# Autodesk Inventor assembly: FO-020.75-NT
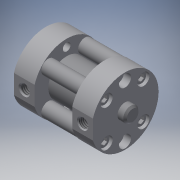
[picture p0: Inventor's stored thumbnail of the model, 180x180]
Saved by Autodesk Inventor 2019.4 (Build 234330000, 330)
## iProperties
Category: PARTsolutions
Company: BIMBA
Created: 2020-02-04
Part Number: FO-020.75-NT
Catalog Web Link: www.cadenas.de
Description: FO, FOD, FOR, FOS-Bimba FLAT-1
Vendor: BIMBA
Document SubType Name: Assembly
Designer: psadmin
Manufacturer: BIMBA
Mass: 12.4329 g
Surface Area: 117.093 cm^2
Volume: 12.4329 cm^3
Density: 1 g/cm^3
PSOL_IDENT_0: {$CADENAS_DATA\23d-libs\bimba\bimba_brand\bimba_imperial\bimba_full_line\flat_cylinders\fo1\bif_asmt
PSOL_IDENT_1: ab.prj},324 {VTYP=3D},{STYP=ASSTAB},{NB=FO-020.75-NT},{LINA=FO-020.75-NT},{NN=FO, FOD, FOR, FOS},{DA
PSOL_IDENT_2: TE=22.01.2020 09:06:06},{GEOMDATE=12.06.2019 07:36:45},{VERSION=},{LINEID=10},{WBVAR=STROKE,ACTING,M
PSOL_IDENT_3: NTR,MNTF,EE,EEL,TWAB,B,RT,LPHD,G,HR,FO,CRB,FS,M,PP,TO,RM,UM,STPT1,STPT3,STPT4,STPTU1,STPTU3,STPTU4,M
PSOL_IDENT_4: RS,W,CB,TB},{WBNUMERIC=STROKE,EEL}  {NB=FO-020.75-NT},{LINA=FO-020.75-NT},{KT=DUMMY},{PN=FO-020.75-N
PSOL_IDENT_5: T},{PNA=(NO ACCESSORIES)},{PNC=FO-020.75-NT},{BORE=9/16\" (02)},{BORE1=0.56250000},{BOREPN=02},{STRO
PSOL_IDENT_6: KE=0.75},{STROKEMIN=0.12500},{STROKEMAX=16.00000000},{ACTING=},{ACTINGALG='','Double Acting, Single
PSOL_IDENT_7: End Rod [FO]', 'D'  , 'Double Acting, Double End Rod [FOD]', 'R', 'Reverse Acting [FOR]', 'S'  ,'Sin
PSOL_IDENT_8: gle Acting [FOS]'},{MNTR=},{MNTF=},{MNT=},{MNTALG='','Standard Counterbored Mounting Holes','1','Piv
PSOL_IDENT_9: ot Mount','1N','Pivot Mount 90 Deg. from Standard','3','Threaded Mounting Holes, Both Ends','3F','Th
PSOL_IDENT_10: readed Mounting Holes, Front','3R','Threaded Mounting Holes, Rear','4','Screw Clearance Holes, Both
PSOL_IDENT_11: Ends','4F','Screw Clearance Holes, Front','4R','Screw Clearance Holes, Rear','5','Nose Mount'},{EEMA
PSOL_IDENT_12: X=17.25},{EE=},{EEALG='','Without Extra Extension','EE','With Extra Extension'},{EEL=0.000},{EELALG=
PSOL_IDENT_13: 0},{OPLALG='','Standard Grease Lube','99','Oil Pre-Lube [99]'},{TWAB=},{TWABALG='','Standard Stainle
PSOL_IDENT_14: ss Steel Body' },{B=},{BALG='','Without Bumper','B','Bumper, Both Ends','BR','Bumper, Rear Only','BF'
PSOL_IDENT_15: ,'Bumper, Front Only'},{RT=NT},{RTALG='', 'Standard Female Thread #8-32 UNC-2B', 'MT', 'Male Rod End
PSOL_IDENT_16: (Fine) #8-32 UNC-2B [MT]', 'NT'  , 'Non-Threaded Rod (Plain Rod) [NT]'},{LPHD=},{LPHDALG='','Standa
PSOL_IDENT_17: rd Pressure Design','D','Low Pressure Hydraulic Design (250 psi max) [D]'},{G=},{GALG='','Standard G
PSOL_IDENT_18: rease Lube','99','Oil Pre-Lube [99]'},{HR=},{HRALG='','N/A'},{HD=},{HDALG='', 'N/A'},{FO=},{FOALG=''
PSOL_IDENT_19: ,'N/A'},{CRB=},{CRBALG='','Standard Rod Bushing','K','Composite Rod Bushing [K]'},{FS=},{FSALG='','S
PSOL_IDENT_20: tandard Friction Seals','L','Low Friction Seals', 'X', 'Ring Rod Seal'},{FSPNL=},{FSPNX=},{M=},{MALG=''
PSOL_IDENT_21: ,'Without Magnetic Position Sensing','M','With Magnetic Position Sensing [M]','M1','With Magnetic Po
PSOL_IDENT_22: sition Sensing (Position 1) [M1]','M3','With Magnetic Position Sensing (Position 3) [M3]' ,'M4','Wit
PSOL_IDENT_23: h Magnetic Position Sensing (Position 4) [M4]' },{PB=},{PBALG='','Standard Body','PB','Composite Bod
PSOL_IDENT_24: y [PB]'},{PP=},{PPALG='','Standard (ports in line, position #1)'},{TO=},{TOALG= '', 'Standard Temp',
PSOL_IDENT_25: 'Q'  , 'Low Temperature Operation (-40°F to 200°F)', 'V'  , 'High Temperature Option (0°F to 400°F)'
PSOL_IDENT_26: },{S=},{SALG='','N/A'},{ST=},{STALG= '' , 'N/A' },{RM=},{RMALG='', 'Chrome Plated Stainless Steel',
PSOL_IDENT_27: 'SR'  , 'Non-Chrome Plated Stainless Steel Rod [SR]'},{UM=},{STPT1=},{STPT1ALG= '' , 'N/A' },{STPT2=
PSOL_IDENT_28: },{STPT2ALG= '' , 'N/A' },{STPT3=},{STPT3ALG= '' , 'N/A' },{STPT4=},{STPT4ALG= '' , 'N/A' },{UMALG= ''
PSOL_IDENT_29: ,'Without Magnetic Position Sensing 90°','U','With Magnetic Position Sensing 90° [U]'  ,'U4','With M
PSOL_IDENT_30: agnetic Position Sensing 90° (Position 4) [U4]' },{STPTU1=},{STPTU1ALG= '' , 'N/A' },{STPTU3=},{STPT
PSOL_IDENT_31: U3ALG= '' , 'N/A' },{STPTU4=},{STPTU4ALG= '' , 'N/A' },{U4ALG= ,'U4','With Magnetic Position Sensing
PSOL_IDENT_32: 90° (Position 4) [U4]' },{SOALG='', 'Without Ring Rod Seal', 'X', 'With Ring Rod Seal'},{SO=},{MRS=
PSOL_IDENT_33: },{MRSALG='','None ','Z','Metallic Rod Scraper [Z]'},{W=},{WALG='', 'Without Wiper', 'W', 'With Wipe
PSOL_IDENT_34: r'},{Y=},{YALG='','N/A'},{RP=},{CB=},{TB=},{A=1.12},{B1=0.13},{BA=0.56},{BA1=0.56},{BB=0.00},{BB1=0.
PSOL_IDENT_35: 69},{BC=0.00},{BD=0.00},{B11=-},{C=0.88},{DD=2},{D=#4},{CPIL=0.12000000},{DC=0.18800000},{DCP=0.1200
PSOL_IDENT_36: 0000},{DCD=0.85500000},{ES=#8-32 UNC-2B},{EC=N/A},{ED=0.460},{F=0.25},{G1=0.14},{H=0.22},{HH=},{J=0.
PSOL_IDENT_37: 34},{K=0.17},{K1=0.17},{K2=0.27},{L=#10-32},{ANGLE=45},{LDP=0.20000000},{LP=0.16000000},{LPDP=0.2800
PSOL_IDENT_38: 0000},{TD=0.65700000},{TDDP=0.10000},{TD1=0.59500},{TD2=0.61000},{TDIN=0.56200},{LSF=0.31250000},{LS
PSOL_IDENT_39: FDP=0.02000000},{BC1=0.81000},{BC2=1.38000},{BC3=1.96000},{BC4=2.52000},{BD1=1.06000},{BD2=1.62000},
PSOL_IDENT_40: {BD3=2.14000},{BD4=2.70000},{BBB=0.56},{FSADD1=0.25000000},{HDADD1=0.13000000},{MADD1=0.875},{M1=0.8
PSOL_IDENT_41: 7500000},{M2=0.62500000},{M3=0.37500000},{RL=1.2},{BL=0.83},{LR=0.63},{FSADD=0},{HDADD=0},{MADD=0},{
PSOL_IDENT_42: ER=},{RL22=0.13},{RL11=0.13000000},{RL1=0.13},{MNTRG=},{MNTRH=},{LG1=0.38000000},{LG=0},{RPART=0.08}
PSOL_IDENT_43: ,{AA1=0.06},{AB1=0.75},{AC1=0.38000000},{AD1=1/2-20 UNF-2A},{AE1=0.498},{AF1=0.31},{MM1=N/A},{MM=-},
PSOL_IDENT_44: {MM2=0.13},{N=-},{N1=N/A},{NN=0.24},{P1=0.000},{NB1=0.00000000},{P=-},{R=-},{R1=#4-40 UNC-2B},{R7=#6
PSOL_IDENT_45: -32 UNC-2B},{Q=-},{Q1=0.19},{S1=-},{S2=0.38},{T=-},{T1=0.19},{U=-},{U1=0.25},{W1=-},{W11=0.75},{X=-}
PSOL_IDENT_46: ,{Y1=-},{Z=-},{AA=-},{AB=-},{AC2=0.00},{AC=-},{AD=-},{AE=-},{AF=-},{Z1=0.19},{Y11=0.63},{X1=0.17},{D
PSOL_IDENT_47: ASH=-},{RTPN1=},{RTPN2=NT},{QPN1=},{QPN2=},{EELPN=},{CBALG='','N/A'},{TBALG='','N/A'},{RPALG='','N/A'
PSOL_IDENT_48: },{CBPN=},{TBPN=},{RPPN=},{STPT1PN=},{STPT2PN=},{STPT3PN=},{STPT4PN=},{RPALG1='','N/A'},{CBALG1='','
PSOL_IDENT_49: N/A'},{TBALG1='','N/A'},{CBPN1=},{TBPN1=},{RPPN1=},{CB1=BC-1},{TB1=-},{RP1=RP-1/2},{LR1=0.63},{PPATH=
PSOL_IDENT_50: fo1_asmtpl.prj},{MNTRALG='','Standard Counterbored Mounting Holes'  ,'1','Pivot Mount','1N','Pivot M
PSOL_IDENT_51: ount 90 Deg. from Standard'   ,'3R','Threaded Mounting Holes, Rear','4R','Screw Clearance Holes, Rea
PSOL_IDENT_52: r','6','F Series Interchange, Counterbored, Rear [6]' ,'7R','F Series Interchange, Threaded, Rear [7
PSOL_IDENT_53: R]'},{MNT2R=},{MNTFALG= '','Standard Counterbored Mounting Holes'       ,'3F','Threaded Mounting Hol
PSOL_IDENT_54: es, Front','4F','Screw Clearance Holes, Front'    ,'5','Nose Mount'      ,'7F','F Series Interchange
PSOL_IDENT_55: , Threaded, Front [7F]'  },{MNT2F=},{MNT5F= ,'5','Nose Mount'  },{MNTPN=},{MNTPNRH=0},{MNTPNRG=0},{W
PSOL_IDENT_56: PN=},{HDPN=},{ASSOPTACC=W},{MATALGHTML=<b>Flat 1 Cylinders:</b><dl><dt>End Caps & Posts:</dt><dd>- A
PSOL_IDENT_57: nodized Aluminum</dd><dt> Seals:</dt><dd>- Buna N </dd><dt>Body:</dt><dd>- 304 Stainless Steel</dd><
PSOL_IDENT_58: dt>Bearings:</dt><dd>- Oil Impregnated Bronze</dd><dt>Rod:</dt><dd>-  303 Stainless Steel</dd></dl>}
PSOL_IDENT_59: ,{STRK2D=0},{X2D=2},{STROKESW=0.750},{EESW=0.000},{FCD=0},{BCD=0},{RCD=0},{CUSTADD=0.0000},{STPTU1PN=
PSOL_IDENT_60: },{STPTU3PN=},{STPTU4PN=},{FOADD=0.000},{NPTF=NT},{OPLPN=},{GPN=},{TU2CFG=},{TU3CFG=},{TU4CFG=},{MNT
PSOL_IDENT_61: 4F=,'4F','Screw Clearance Holes, Front'},{NPT=-},{HHFT=0.12},{HHCF=N/A},{HHMT=N/A},{HHMTH=N/A},{HHNP
PSOL_IDENT_62: T=N/A},{FTL1=0.460},{NEWPRA=1}
NN: 0.24
NT: Bimba FLAT-1
NB: FO-020.75-NT
NBSYN: $PNC.
LINA: FO-020.75-NT
PN: FO-020.75-NT
PNA: (NO ACCESSORIES)
BORE: 9/16" (02)
STROKE: 0.75
ACTING: Double Acting, Single End Rod [FO]
MNTR: Standard Counterbored Mounting Holes
MNTF: Standard Counterbored Mounting Holes
EE: Standard Rod Extension
EEL: 0
TWAB: Standard Stainless Steel Body
B: Without Bumper
RT: Non-Threaded Rod (Plain Rod) [NT]
LPHD: Standard Pressure Design
G: Standard Grease Lube
HR: N/A
FO: N/A
CRB: Standard Rod Bushing
FS: Standard O-Ring Seals
M: Without Magnetic Position Sensing
PP: Standard (ports in line, position #1)
TO: Standard -20° to 200°F (-29° to 95°C)
RM: Chrome Plated Stainless Steel
UM: Without Magnetic Position Sensing 90°
STPT1: N/A
STPT3: N/A
STPT4: N/A
STPTU1: N/A
STPTU3: N/A
STPTU4: N/A
W: Without Wiper
CB: N/A
TB: N/A
A: 1.12
B1: 0.13
BA: 0.56
BB: 0
BC: 0
BD: 0
B11: -
C: 0.88
DD: 2
D: #4
ES: #8-32 UNC-2B
EC: N/A
ED: 0.46
F: 0.25
G1: 0.14
H: 0.22
J: 0.34
K: 0.17
L: #10-32
MM: -
MM2: 0.13
N: -
P: -
R: -
Q: -
S1: -
T: -
U: -
W1: -
X: -
Y1: -
Z: -
AA: -
AB: -
AC: -
AD: -
AE: -
AF: -
SUPPLIER: BIMBA
ARTICLENO: FO-020.75-NT
BOMINFO: FO-020.75-NT
CREATOR: CADENAS GmbH
Title: FO-020.75-NT
Author: Cadenas PARTsolutions
Comments: Bimba FLAT-1
## Documents named in this file (8)
- T:\EIT\2020 Infinite Recharge\2020 ROBOT\COMMON PARTS\AIR CYLINDERS\FO-020.75-NT\AIS2018\FO-020_75-NT.iam
- T:\EIT\2020 Infinite Recharge\2020 ROBOT\COMMON PARTS\AIR CYLINDERS\FO-020.75-NT\AIS2018\02-2-0_125-FO1_BM_heads_left-bif.ipt
- T:\EIT\2020 Infinite Recharge\2020 ROBOT\COMMON PARTS\AIR CYLINDERS\FO-020.75-NT\AIS2018\020_825-FO1_BM_tube.ipt
- T:\EIT\2020 Infinite Recharge\2020 ROBOT\COMMON PARTS\AIR CYLINDERS\FO-020.75-NT\AIS2018\02-1NT-0_125-FO1_BM_heads-bif.ipt
- T:\EIT\2020 Infinite Recharge\2020 ROBOT\COMMON PARTS\AIR CYLINDERS\FO-020.75-NT\AIS2018\D-D0144-SS-1-bif.ipt
- T:\EIT\2020 Infinite Recharge\2020 ROBOT\COMMON PARTS\AIR CYLINDERS\FO-020.75-NT\AIS2018\POST0_5625-0_625-bif.ipt
- T:\EIT\2020 Infinite Recharge\2020 ROBOT\COMMON PARTS\AIR CYLINDERS\FO-020.75-NT\AIS2018\FO-020_751_194NT-00_rod-bif.ipt
- T:\EIT\2020 Infinite Recharge\2020 ROBOT\COMMON PARTS\AIR CYLINDERS\FO-020.75-NT\AIS2018\0_56250_075-rod_part0.ipt
## Components (13 placed, 7 different names)
1. 02-2-0_125-FO1_BM_heads_left-bif:1
2. 020_825-FO1_BM_tube:1
3. 02-1NT-0_125-FO1_BM_heads-bif:1 — Insert:2
4. D-D0144-SS-1-bif:1
5. D-D0144-SS-1-bif:2
6. D-D0144-SS-1-bif:3
7. D-D0144-SS-1-bif:4
8. POST0_5625-0_625-bif:1
9. POST0_5625-0_625-bif:2
10. POST0_5625-0_625-bif:3
11. POST0_5625-0_625-bif:4
12. FO-020_751_194NT-00_rod-bif:1 — Insert:1
13. 0_56250_075-rod_part0:1 — Insert:1, Insert:2
## Relationships (2: Insert 2)
- Insert:1: FO-020_751_194NT-00_rod-bif:1 ↔ 0_56250_075-rod_part0:1
- Insert:2: 02-1NT-0_125-FO1_BM_heads-bif:1 ↔ 0_56250_075-rod_part0:1
